# Autodesk Inventor assembly: workbench
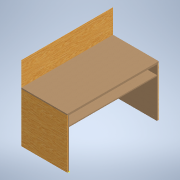
[picture p0: Inventor's stored thumbnail of the model, 180x180]
Saved by Autodesk Inventor 2022 (Build 260153000, 153)
## iProperties
Created: 2022-02-21
Part Number: workbench
Document SubType Name: Assembly
Designer: MarkP
Author: MarkP
## Documents named in this file (9)
- C:\Users\MarkP\Documents\Mark\final\workbench.iam
- C:\Users\MarkP\Documents\Mark\final\desk.ipt
- C:\Users\MarkP\Documents\Mark\final\wallL1.ipt
- C:\Users\MarkP\Documents\Mark\final\wallL2.ipt
- C:\Users\MarkP\Documents\Mark\final\wallL1_MIR.ipt
- C:\Users\MarkP\Documents\Mark\final\wallL2_MIR.ipt
- C:\Users\MarkP\Documents\Mark\final\basedraws.ipt
- C:\Users\MarkP\Documents\Mark\final\reardraws.ipt
- C:\Users\MarkP\Documents\Mark\final\backboard.ipt
## Components (8 placed, 8 different names)
1. desk:1 — Mate:2, Flush:3, Mate:3, Flush:6, Mate:7, Mate:9, Flush:9
2. wallL1:1 — Flush:1, Mate:1, Flush:2, Flush:3, Flush:7, Mate:8
3. wallL2:1 — Flush:1, Mate:1, Flush:2, Mate:2, Mate:3, Mate:6, Flush:8
4. wallL1_MIR:1 — Flush:4, Mate:4, Flush:5
5. wallL2_MIR:1 — Flush:4, Mate:4, Flush:5, Mate:5
6. basedraws:1 — Flush:6, Mate:5, Flush:7
7. reardraws:1 — Mate:6, Mate:7, Mate:8
8. backboard:1 — Mate:9, Flush:8, Flush:9
## Relationships (18: Flush 9, Mate 9)
- Flush:1: wallL1:1 ↔ wallL2:1
- Mate:1: wallL1:1 ↔ wallL2:1
- Flush:2: wallL1:1 ↔ wallL2:1
- Mate:2: desk:1 ↔ wallL2:1
- Flush:3: desk:1 ↔ wallL1:1
- Mate:3: desk:1 ↔ wallL2:1
- Flush:4: wallL1_MIR:1 ↔ wallL2_MIR:1
- Mate:4: wallL1_MIR:1 ↔ wallL2_MIR:1
- Flush:5: wallL1_MIR:1 ↔ wallL2_MIR:1
- Flush:6: desk:1 ↔ basedraws:1
- Mate:5: wallL2_MIR:1 ↔ basedraws:1
- Flush:7: wallL1:1 ↔ basedraws:1
- Mate:6: wallL2:1 ↔ reardraws:1
- Mate:7: desk:1 ↔ reardraws:1
- Mate:8: wallL1:1 ↔ reardraws:1
- Mate:9: desk:1 ↔ backboard:1
- Flush:8: wallL2:1 ↔ backboard:1
- Flush:9: desk:1 ↔ backboard:1
